# Autodesk Inventor assembly: GEA MOTION
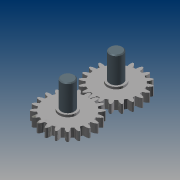
[picture p0: Inventor's stored thumbnail of the model, 180x180]
Saved by Autodesk Inventor 2014 (Build 180170000, 170)
## iProperties
Created: 2021-03-18
Part Number: GEA MOTION
Document SubType Name: Assembly
Designer: Think Station
Author: Think Station
## Documents named in this file (3)
- E:\Entraco_Diptanshu\3D\##TEST##\Gear Animation\GEAR MOTION.iam
- E:\Entraco_Diptanshu\3D\##TEST##\Gear Animation\Part1.ipt
- E:\Entraco_Diptanshu\3D\##TEST##\Gear Animation\Shaft.ipt
## Components (4 placed, 2 different names)
1. Part1:1 — Insert:1, Mate:3, Rotation:1
2. Shaft:1 — Mate:1, Mate:2, Insert:1, Mate:3, Flush:1
3. Part1:2 — Rotation:1
4. Shaft:2 — Mate:5, Flush:1, Mate:6, Angle:1
## Relationships (11: Mate 6, Insert 2, Flush 1, RelateRotation 1, Angle 1)
- Mate:1: Shaft:1
- Mate:2: Shaft:1
- Insert:1: Part1:1 ↔ Shaft:1
- Mate:3: Part1:1 ↔ Shaft:1
- [Insert]: Part1:2 ↔ Shaft:2
- [Mate]: Part1:2 ↔ Shaft:2
- Mate:5 (112 mm): Shaft:2
- Flush:1: Shaft:1 ↔ Shaft:2
- Mate:6: Shaft:2
- Rotation:1 [RelateRotation] (1 ul): Part1:1 ↔ Part1:2
- Angle:1 (1080 deg): Shaft:2
## Named parameters: d7_d5 = 0 mm, d8_d6 = 0 mm
